# Autodesk Inventor assembly: fan_3007
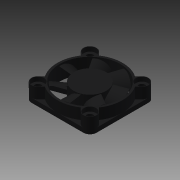
[picture p0: Inventor's stored thumbnail of the model, 180x180]
Saved by Autodesk Inventor 2013 (Build 170138000, 138)
## iProperties
Created: 2014-03-19
Part Number: fan_3007
Document SubType Name: Assembly
Designer: Noa Izumi
Control State: 0
Master: False
Checked Out: False
Shininess: 20.0
Density: 0.0
Volumn: 0.0
Area: 0.0
PropertySet Name: Model Information
Author: Noa Izumi
## Documents named in this file (3)
- C:\reprap\reprap_13\fan_3007.iam
- C:\reprap\reprap_13\fan_3007_base.ipt
- C:\reprap\reprap_13\fan_3007_blaze.ipt
## Components (2 placed, 2 different names)
1. fan_3007_base:1 — 插入:1
2. fan_3007_blaze:1 — 插入:1
## Relationships (1: Insert 1)
- 插入:1 [Insert]: fan_3007_base:1 ↔ fan_3007_blaze:1
